# Autodesk Inventor assembly: assembly
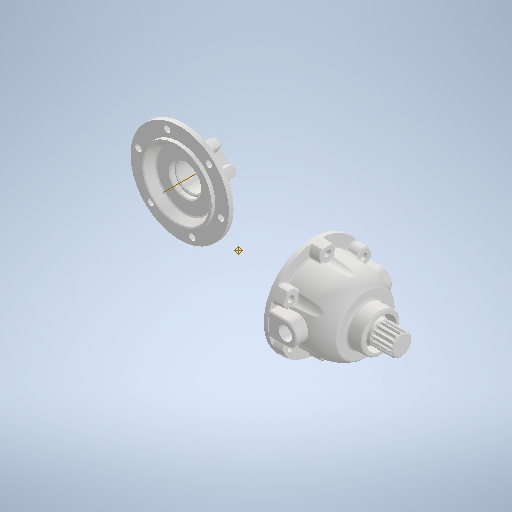
[picture p0: Inventor's stored thumbnail of the model, 512x512]
Saved by Autodesk Inventor 2025.2 (Build 292293000, 293)
## iProperties
Created: 2025-06-12
Part Number: assembly
Document SubType Name: Assembly
Designer: Kacper
Author: Kacper
## Documents named in this file (5)
- D:\studia\semestr 4\Grafika inżynierska\Projekt 4\assembly.iam
- D:\studia\semestr 4\Grafika inżynierska\Projekt 4\housing.ipt
- D:\studia\semestr 4\Grafika inżynierska\Projekt 4\spacer_washer.ipt
- D:\studia\semestr 4\Grafika inżynierska\Projekt 4\rear_cover.ipt
- D:\studia\semestr 4\Grafika inżynierska\Projekt 4\bevel_gear_2.ipt
## Components (4 placed, 4 different names)
1. housing:1 — Mate:5, Mate:8
2. rear_cover:1
3. spacer_washer:1 — Mate:6, Mate:7, Mate:8
4. bevel_gear_2:1 — Mate:5, Mate:6, Mate:7
## Relationships (4: Mate 4)
- Mate:5: housing:1 ↔ bevel_gear_2:1
- Mate:6: spacer_washer:1 ↔ bevel_gear_2:1
- Mate:7: spacer_washer:1 ↔ bevel_gear_2:1
- Mate:8: housing:1 ↔ spacer_washer:1
